# Autodesk Inventor assembly: Front_10Gbit_CAM_Assembly
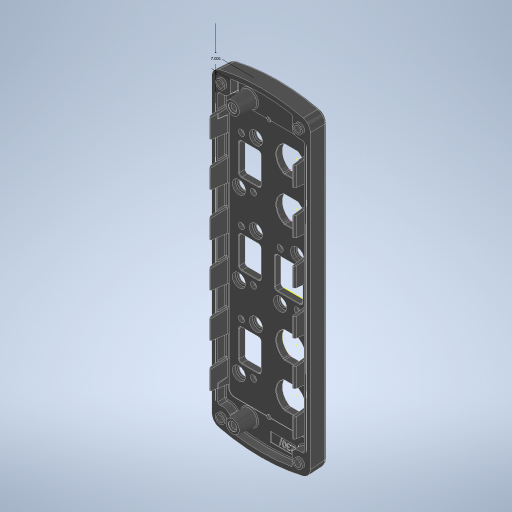
[picture p0: Inventor's stored thumbnail of the model, 512x512]
Saved by Autodesk Inventor 2024.2 (Build 282272000, 272)
## iProperties
Created: 2024-03-08
Part Number: Front_10Gbit_CAM_Assembly
Document SubType Name: Assembly
Designer: lgnds
Author: lgnds
## Documents named in this file (4)
- C:\Users\lgnds\Documents\GitHub\REACH-Hardware\CAD\InventorProject\Manufacturing\Front_10Gbit_CAM_Assembly.iam
- C:\Users\lgnds\Documents\GitHub\REACH-Hardware\CAD\InventorProject\Manufacturing\PanelJig.ipt
- C:\Users\lgnds\Documents\GitHub\REACH-Hardware\CAD\InventorProject\Front_Panel\Panel\1009799_3D.ipt
- C:\Users\lgnds\Documents\GitHub\REACH-Hardware\CAD\InventorProject\Front_Panel\Panel\1009799_3D_Front_10Gbit.ipt
## Components (5 placed, 3 different names)
1. PanelJig:1 — Rigid:1, Rigid:2, Rigid:3, Rigid:4
2. 1009799_3D:1 — Rigid:1
3. 1009799_3D_Front_10Gbit:1 — Rigid:2
4. 1009799_3D:2 — Rigid:3
5. 1009799_3D_Front_10Gbit:2 — Rigid:4
## Relationships (4: WeldJoint 4)
- Rigid:1 [WeldJoint]: PanelJig:1 ↔ 1009799_3D:1
- Rigid:2 [WeldJoint]: PanelJig:1 ↔ 1009799_3D_Front_10Gbit:1
- Rigid:3 [WeldJoint]: PanelJig:1 ↔ 1009799_3D:2
- Rigid:4 [WeldJoint]: PanelJig:1 ↔ 1009799_3D_Front_10Gbit:2
